# Autodesk Inventor assembly: Sensor Modul
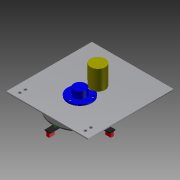
[picture p0: Inventor's stored thumbnail of the model, 180x180]
Saved by Autodesk Inventor 2014 (Build 180170000, 170)
## iProperties
Created: 2014-02-18
Part Number: Sensor Modul
Document SubType Name: Assembly
Designer: Pinkponk
Author: Pinkponk
## Documents named in this file (10)
- X:\Projekt\Min Robot\Min Robot\Sensor Modul.iam
- X:\Projekt\Min Robot\Min Robot\SensorPlatta.ipt
- X:\Projekt\Min Robot\Min Robot\Släpring.ipt
- X:\Projekt\Min Robot\Min Robot\Kugghjul 5mm.ipt
- X:\Projekt\Min Robot\Min Robot\Motor Sensor.ipt
- X:\Projekt\Min Robot\Min Robot\Kugghjul 4mm.ipt
- X:\Projekt\Min Robot\Min Robot\SensorSkiva Plugg.ipt
- X:\Projekt\Min Robot\Min Robot\Skiva.ipt
- X:\Projekt\Min Robot\Min Robot\Sensor.ipt
- X:\Projekt\Min Robot\Min Robot\Sensor Avstånd.ipt
## Components (12 placed, 9 different names)
1. SensorPlatta:1 — Insert:1, Insert:3
2. Släpring:1 — Insert:1, Insert:2, Insert:5
3. Kugghjul 5mm:1 — Insert:2
4. Motor Sensor:1 — Insert:3, Insert:4
5. Kugghjul 4mm:1 — Insert:4
6. SensorSkiva Plugg:1 — Insert:5, Insert:6
7. Skiva:1 — Insert:6, Insert:8
8. Sensor Avstånd:1 — Insert:7, Insert:8
9. Sensor:1 — Insert:7
10. Sensor:2
11. Sensor:3
12. Sensor:4
## Component patterns: (4 elements, first: Sensor:1)
## Relationships (8: Insert 8)
- Insert:1: SensorPlatta:1 ↔ Släpring:1
- Insert:2: Släpring:1 ↔ Kugghjul 5mm:1
- Insert:3: SensorPlatta:1 ↔ Motor Sensor:1
- Insert:4: Motor Sensor:1 ↔ Kugghjul 4mm:1
- Insert:5 (2 mm): Släpring:1 ↔ SensorSkiva Plugg:1
- Insert:6: SensorSkiva Plugg:1 ↔ Skiva:1
- Insert:7: Sensor Avstånd:1 ↔ Sensor:1
- Insert:8: Skiva:1 ↔ Sensor Avstånd:1
